# Autodesk Inventor assembly: iLMbot V3 75%
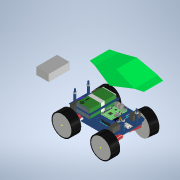
[picture p0: Inventor's stored thumbnail of the model, 180x180]
Saved by Autodesk Inventor 2021 (Build 250183000, 183)
## iProperties
Company: none
Created: 2021-02-18
Part Number: iLMbot V3 75%
Description: CATIA V5 STEP Exchange
Document SubType Name: Assembly
Designer: Ashiqrahman
Authority: none
Sending System: Autodesk Inventor 2021
Preprocessor: ST-DEVELOPER v18.1
Title: D:\LM bot\iLMbot V3 75%.stp
Author: ASUS
## Documents named in this file (31)
- D:\Projects\P_Intelligent Line Marking Bot\Design\LMBOT V3 80%\iLMbot V3 75%.iam
- D:\Projects\P_Intelligent Line Marking Bot\Design\LMBOT V3 80%\chasis.ipt
- D:\Projects\P_Intelligent Line Marking Bot\Design\LMBOT V3 80%\Part2.ipt
- D:\Projects\P_Intelligent Line Marking Bot\Design\LMBOT V3 80%\MG-958 servo.iam
- D:\Projects\P_Intelligent Line Marking Bot\Design\LMBOT V3 80%\knucle.ipt
- D:\Projects\P_Intelligent Line Marking Bot\Design\LMBOT V3 80%\Symmetry of JGB37-520.iam
- D:\Projects\P_Intelligent Line Marking Bot\Design\LMBOT V3 80%\Document.ipt
- D:\Projects\P_Intelligent Line Marking Bot\Design\LMBOT V3 80%\Symmetry of Document.ipt
- D:\Projects\P_Intelligent Line Marking Bot\Design\LMBOT V3 80%\Symmetry of Symmetry of Document.ipt
- D:\Projects\P_Intelligent Line Marking Bot\Design\LMBOT V3 80%\Part1.ipt
- D:\Projects\P_Intelligent Line Marking Bot\Design\LMBOT V3 80%\n20 geared motor.ipt
- D:\Projects\P_Intelligent Line Marking Bot\Design\LMBOT V3 80%\8mm flange nut.ipt
- D:\Projects\P_Intelligent Line Marking Bot\Design\LMBOT V3 80%\M6-lead screw.ipt
- D:\Projects\P_Intelligent Line Marking Bot\Design\LMBOT V3 80%\wheel.ipt
- D:\Projects\P_Intelligent Line Marking Bot\Design\LMBOT V3 80%\MG-958 servo_MIR.iam
- D:\Projects\P_Intelligent Line Marking Bot\Design\LMBOT V3 80%\knucle_MIR.ipt
- D:\Projects\P_Intelligent Line Marking Bot\Design\LMBOT V3 80%\Symmetry of JGB37-520_MIR.iam
- D:\Projects\P_Intelligent Line Marking Bot\Design\LMBOT V3 80%\wheel_MIR.ipt
- D:\Projects\P_Intelligent Line Marking Bot\Design\LMBOT V3 80%\MG-958 servo_MIR1.iam
- D:\Projects\P_Intelligent Line Marking Bot\Design\LMBOT V3 80%\knucle_MIR1.ipt
- D:\Projects\P_Intelligent Line Marking Bot\Design\LMBOT V3 80%\Symmetry of JGB37-520_MIR1.iam
- D:\Projects\P_Intelligent Line Marking Bot\Design\LMBOT V3 80%\wheel_MIR1.ipt
- D:\Projects\P_Intelligent Line Marking Bot\Design\LMBOT V3 80%\MG-958 servo_MIR_MIR.iam
- D:\Projects\P_Intelligent Line Marking Bot\Design\LMBOT V3 80%\Symmetry of JGB37-520_MIR_MIR.iam
- D:\Projects\P_Intelligent Line Marking Bot\Design\LMBOT V3 80%\wheel_MIR_MIR.ipt
- D:\Projects\A_Electronics CAD model\arduino-mega-atmega-2560-1.snapshot.3\Arduino Mega ATmega 2560.iam
- D:\Projects\A_Electronics CAD model\raspberry-pi-27.snapshot.7\RaspberryPi.iam
- C:\Users\techv\Documents\C drive Inventor Files\motor driver.ipt
- D:\Projects\P_Intelligent Line Marking Bot\Design\LMBOT V3 80%\Li-ion 12 volt.ipt
- D:\Projects\A_Electronics CAD model\ublox-gps-1.snapshot.1\gps\parts\GPS_ublox_board.ipt
- D:\Projects\A_Electronics CAD model\mpu-9250-9dof-imu-1.snapshot.4\MPU-9250.iam
## Components (43 placed, 31 different names)
1. chasis — Mate:1, Flush:1, Flush:2, Mate:2, Flush:3, Flush:4, Mate:9, Mate:10, Flush:13, Mate:11, Mate:12, Mate:13, Mate:14, Mate:15, Mate:16, Flush:18, Mate:20, Mate:21, Mate:23, Mate:24, Mate:25, Mate:26, Mate:27, Mate:28, Mate:29, Mate:30, Mate:31
2. Part2.1
3. MG-958 servo.2 [sub-assembly] — Mate:29, Mate:30, Mate:31, Mate:38, Mate:44
4. knucle.1
5. Symmetry of JGB37-520.1.2 [sub-assembly]
6. Document.1
7. Symmetry of Document.1.1
8. Symmetry of Symmetry of Document.1.1.1
9. Symmetry of Document.1.2
10. Part1:2
11. n20 geared motor:2
12. 8mm flange nut:2
13. M6-lead screw:1
14. wheel:1
15. MG-958 servo_MIR:1 [sub-assembly] — Mate:27, Mate:28, Mate:39, Mate:43
16. knucle_MIR:1
17. Symmetry of JGB37-520_MIR:1 [sub-assembly]
18. wheel_MIR:1
19. MG-958 servo_MIR1:1 [sub-assembly] — Mate:23, Mate:24, Mate:40, Mate:45
20. knucle_MIR1:1 — Mate:17, Mate:22, Mate:40, Mate:45
21. Symmetry of JGB37-520_MIR1:1 [sub-assembly] — Mate:17, Mate:22, Mate:54, Mate:55
22. wheel_MIR1:1
23. MG-958 servo_MIR_MIR:1 [sub-assembly] — Mate:25, Mate:26, Mate:41, Mate:42
24. Symmetry of JGB37-520_MIR_MIR:1 [sub-assembly] — Mate:8
25. wheel_MIR_MIR:1 — Mate:8, Mate:46, Mate:51
26. Arduino Mega ATmega 2560:1 [sub-assembly] — Mate:1, Flush:1, Flush:2
27. RaspberryPi:1 [sub-assembly] — Mate:2, Flush:3, Flush:4
28. Li-ion 12 volt:1 — Mate:9
29. GPS_ublox_board:1 — Mate:10, Flush:13, Mate:13, Mate:14, Mate:15, Mate:16
30. MPU-9250:1 [sub-assembly] — Mate:11, Mate:12
31. motor driver:2 — Mate:18, Flush:14, Flush:15, Flush:20, Flush:21, Mate:21
32. motor driver:3 — Mate:19, Flush:16, Flush:17, Mate:20, Flush:20, Flush:21
33. motor driver:4 — Mate:18, Flush:14, Flush:15
34. motor driver:5 — Mate:19, Flush:16, Flush:17, Flush:19
35. knucle_MIR1:2 — Mate:41, Mate:42
36. Symmetry of JGB37-520_MIR1:2 [sub-assembly] — Mate:46, Mate:51
37. knucle_MIR1:3 — Mate:39, Mate:43
38. Symmetry of JGB37-520_MIR1:3 [sub-assembly] — Mate:47, Mate:50
39. knucle_MIR1:4 — Mate:38, Mate:44
40. Symmetry of JGB37-520_MIR1:4 [sub-assembly] — Mate:52, Mate:53
41. wheel_MIR_MIR:2 — Mate:52, Mate:53
42. wheel_MIR_MIR:3 — Mate:47, Mate:50
43. wheel_MIR_MIR:4 — Mate:54, Mate:55
## Relationships (61: Mate 48, Flush 13)
- Mate:1: chasis ↔ Arduino Mega ATmega 2560:1
- Flush:1 (65 mm): chasis ↔ Arduino Mega ATmega 2560:1
- Flush:2 (10 mm): chasis ↔ Arduino Mega ATmega 2560:1
- Mate:2: chasis ↔ RaspberryPi:1
- Flush:3 (15 mm): chasis ↔ RaspberryPi:1
- Flush:4 (15 mm): chasis ↔ RaspberryPi:1
- Mate:8: Symmetry of JGB37-520_MIR_MIR:1 ↔ wheel_MIR_MIR:1
- Mate:9: chasis ↔ Li-ion 12 volt:1
- Mate:10: chasis ↔ GPS_ublox_board:1
- Flush:13 (10 mm): chasis ↔ GPS_ublox_board:1
- Mate:11: chasis ↔ MPU-9250:1
- Mate:12: chasis ↔ MPU-9250:1
- Mate:13: chasis ↔ GPS_ublox_board:1
- Mate:14: chasis ↔ GPS_ublox_board:1
- Mate:15: chasis ↔ GPS_ublox_board:1
- Mate:16: chasis ↔ GPS_ublox_board:1
- Mate:17: knucle_MIR1:1 ↔ Symmetry of JGB37-520_MIR1:1
- Mate:18: motor driver:2 ↔ motor driver:4
- Flush:14: motor driver:2 ↔ motor driver:4
- Flush:15: motor driver:2 ↔ motor driver:4
- Mate:19: motor driver:3 ↔ motor driver:5
- Flush:16: motor driver:3 ↔ motor driver:5
- Flush:17: motor driver:3 ↔ motor driver:5
- Flush:18 (25 mm): chasis
- Mate:20: chasis ↔ motor driver:3
- Flush:19: motor driver:5
- Flush:20: motor driver:2 ↔ motor driver:3
- Flush:21: motor driver:2 ↔ motor driver:3
- Mate:21: chasis ↔ motor driver:2
- Mate:22: knucle_MIR1:1 ↔ Symmetry of JGB37-520_MIR1:1
- Mate:23: chasis ↔ MG-958 servo_MIR1:1
- Mate:24: chasis ↔ MG-958 servo_MIR1:1
- Mate:25: chasis ↔ MG-958 servo_MIR_MIR:1
- Mate:26: chasis ↔ MG-958 servo_MIR_MIR:1
- Mate:27: chasis ↔ MG-958 servo_MIR:1
- Mate:28: chasis ↔ MG-958 servo_MIR:1
- Mate:29: chasis ↔ MG-958 servo.2
- Mate:30: chasis ↔ MG-958 servo.2
- Mate:31: chasis ↔ MG-958 servo.2
- [Mate]: knucle_MIR1:2 ↔ Symmetry of JGB37-520_MIR1:2
- [Mate]: knucle_MIR1:2 ↔ Symmetry of JGB37-520_MIR1:2
- [Mate]: knucle_MIR1:3 ↔ Symmetry of JGB37-520_MIR1:3
- [Mate]: knucle_MIR1:3 ↔ Symmetry of JGB37-520_MIR1:3
- [Mate]: knucle_MIR1:4 ↔ Symmetry of JGB37-520_MIR1:4
- [Mate]: knucle_MIR1:4 ↔ Symmetry of JGB37-520_MIR1:4
- Mate:38: MG-958 servo.2 ↔ knucle_MIR1:4
- Mate:39: MG-958 servo_MIR:1 ↔ knucle_MIR1:3
- Mate:40: MG-958 servo_MIR1:1 ↔ knucle_MIR1:1
- Mate:41: MG-958 servo_MIR_MIR:1 ↔ knucle_MIR1:2
- Mate:42: MG-958 servo_MIR_MIR:1 ↔ knucle_MIR1:2
- Mate:43: MG-958 servo_MIR:1 ↔ knucle_MIR1:3
- Mate:44: MG-958 servo.2 ↔ knucle_MIR1:4
- Mate:45: MG-958 servo_MIR1:1 ↔ knucle_MIR1:1
- Mate:46: wheel_MIR_MIR:1 ↔ Symmetry of JGB37-520_MIR1:2
- Mate:47: Symmetry of JGB37-520_MIR1:3 ↔ wheel_MIR_MIR:3
- Mate:50: Symmetry of JGB37-520_MIR1:3 ↔ wheel_MIR_MIR:3
- Mate:51: wheel_MIR_MIR:1 ↔ Symmetry of JGB37-520_MIR1:2
- Mate:52: Symmetry of JGB37-520_MIR1:4 ↔ wheel_MIR_MIR:2
- Mate:53: Symmetry of JGB37-520_MIR1:4 ↔ wheel_MIR_MIR:2
- Mate:54: Symmetry of JGB37-520_MIR1:1 ↔ wheel_MIR_MIR:4
- Mate:55: Symmetry of JGB37-520_MIR1:1 ↔ wheel_MIR_MIR:4
## Named parameters: d57_d47 = 0 mm, d58_d33 = 0 mm, d59_d47 = 0 mm, d60_d33 = 0 mm, d61_d47 = 0 mm, d62_d33 = 0 mm
